# Autodesk Inventor assembly: ensamble_general
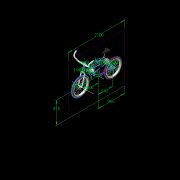
[picture p0: Inventor's stored thumbnail of the model, 180x180]
Saved by Autodesk Inventor 2021 (Build 250183000, 183)
## iProperties
Created: 2021-04-10
Part Number: ensamble_general
Document SubType Name: Assembly
Designer: j2seb
Author: j2seb
## Documents named in this file (10)
- C:\Users\maaro\Documents\UNAL\Automatización de Procesos de Manufactura\Github\Proyecto_APM\02 Inventor\ensamble_general.iam
- C:\Users\maaro\Documents\UNAL\Automatización de Procesos de Manufactura\Github\Proyecto_APM\02 Inventor\Marco_Bicicleta.iam
- C:\Users\maaro\Documents\UNAL\Automatización de Procesos de Manufactura\Github\Proyecto_APM\02 Inventor\Manubrio.ipt
- C:\Users\maaro\Documents\UNAL\Automatización de Procesos de Manufactura\Github\Proyecto_APM\02 Inventor\Ensamble_Llanta.iam
- C:\Users\maaro\Documents\UNAL\Automatización de Procesos de Manufactura\Github\Proyecto_APM\02 Inventor\sillin.iam
- C:\Users\maaro\Documents\UNAL\Automatización de Procesos de Manufactura\Github\Proyecto_APM\02 Inventor\Transmision\Design Accelerator\Roller Chain Sprocket11.ipt
- C:\Users\maaro\Documents\UNAL\Automatización de Procesos de Manufactura\Github\Proyecto_APM\02 Inventor\Transmision\Design Accelerator\Roller Chain Sprocket21.ipt
- C:\Users\maaro\Documents\UNAL\Automatización de Procesos de Manufactura\Github\Proyecto_APM\02 Inventor\Transmision\Design Accelerator\Roller Chain1.ipt
- C:\Users\maaro\Documents\UNAL\Automatización de Procesos de Manufactura\Github\Proyecto_APM\02 Inventor\Transmision\Eslabón 1.ipt
- C:\Users\maaro\Documents\UNAL\Automatización de Procesos de Manufactura\Github\Proyecto_APM\02 Inventor\Transmision\Eslabón 2.ipt
## Components (122 placed, 9 different names)
1. Marco_Bicicleta:1 [sub-assembly] — Coincidencia:2, Coincidencia:3, Flush:1, Cylindrical:2, Mate:5, Mate:6, Mate:8, Mate:10
2. Manubrio:1 — Flush:1, Cylindrical:3, Mate:7, Mate:8
3. Ensamble_Llanta:1 [sub-assembly] — Coincidencia:2
4. Ensamble_Llanta:2 [sub-assembly] — Cylindrical:3
5. sillin:1 [sub-assembly] — Cylindrical:2, Mate:5
6. Roller Chain Sprocket1:1 — Mate:14, Mate:16
7. Roller Chain Sprocket2:1 — Mate:13, Mate:15
8. Roller Chain:1 — Mate:9, Mate:11, Mate:12, Mate:15, Mate:16, Mate:17, Transitional:1, Transitional:2, Transitional:3, Transitional:4, Transitional:5, Transitional:7, Transitional:8, Transitional:9, Transitional:10, Transitional:11, Transitional:12, Transitional:13, Transitional:14, Transitional:15, Transitional:16, Transitional:17, Transitional:18, Transitional:19, Transitional:20, Transitional:21, Transitional:22, Transitional:23, Transitional:24, Transitional:25, Transitional:26, Transitional:27, Transitional:28, Transitional:29, Transitional:30, Transitional:31, Transitional:32, Transitional:33, Transitional:34, Transitional:35, Transitional:36, Transitional:37, Transitional:38, Transitional:39, Transitional:40, Transitional:41, Transitional:42, Transitional:43, Transitional:44, Transitional:45, Transitional:46, Transitional:47, Transitional:48, Transitional:49, Transitional:50, Transitional:51, Transitional:52, Transitional:53, Transitional:54, Transitional:55, Transitional:56, Transitional:57, Transitional:58, Transitional:59, Transitional:60, Transitional:61, Transitional:62, Transitional:63, Transitional:64, Transitional:65, Transitional:66, Transitional:67, Transitional:68, Transitional:69, Transitional:70, Transitional:71, Transitional:72, Transitional:73, Transitional:74, Transitional:75, Transitional:76, Transitional:77, Transitional:78, Transitional:79, Transitional:80, Transitional:81, Transitional:82, Transitional:83, Transitional:84, Transitional:85, Transitional:86, Transitional:87, Transitional:88, Transitional:89, Transitional:90, Transitional:91, Transitional:92, Transitional:93, Transitional:94, Transitional:95, Transitional:96, Transitional:97, Transitional:98, Transitional:99, Transitional:100, Transitional:101, Transitional:102, Transitional:103, Transitional:104, Transitional:105, Transitional:106, Transitional:107, Transitional:108, Transitional:109, Transitional:110, Transitional:111, Transitional:112, Transitional:113, Transitional:114, Transitional:115, Transitional:116, Transitional:117
9. Eslabón 1:1 — Mate:17, Transitional:1, Transitional:2, Mate:18, Mate:19, Mate:20, Mate:21, Mate:22
10. Eslabón 2:1 — Mate:18, Mate:19
11. Eslabón 1:2 — Mate:22, Transitional:3, Transitional:4, Mate:23, Mate:24, Mate:25
12. Eslabón 2:2 — Mate:20, Mate:21, Mate:23
13. Eslabón 1:3 — Mate:26, Transitional:5, Mate:27, Mate:29, Transitional:117
14. Eslabón 2:3 — Mate:24, Mate:25, Mate:26, Mate:27, Mate:28, Mate:30
15. Eslabón 1:4 — Mate:30, Transitional:7, Transitional:8, Mate:31, Mate:33, Transitional:9
16. Eslabón 2:4 — Mate:28, Mate:29, Mate:31, Mate:32
17. Eslabón 1:5 — Mate:34, Transitional:10, Transitional:11, Mate:35, Mate:37
18. Eslabón 2:5 — Mate:32, Mate:33, Mate:34, Mate:35, Mate:36
19. Eslabón 1:6 — Mate:38, Transitional:12, Transitional:13, Mate:39, Mate:41, Transitional:14
20. Eslabón 2:6 — Mate:36, Mate:37, Mate:38, Mate:39, Mate:40
21. Eslabón 1:7 — Mate:42, Transitional:15, Transitional:16, Mate:43, Mate:45
22. Eslabón 2:7 — Mate:40, Mate:41, Mate:42, Mate:43, Mate:44
23. Eslabón 1:8 — Mate:46, Transitional:17, Transitional:18, Mate:47, Mate:49
24. Eslabón 2:8 — Mate:44, Mate:45, Mate:46, Mate:47, Mate:48
25. Eslabón 1:9 — Mate:50, Transitional:19, Transitional:20, Mate:51, Mate:53
26. Eslabón 2:9 — Mate:48, Mate:49, Mate:50, Mate:51, Mate:52
27. Eslabón 1:10 — Mate:54, Transitional:21, Transitional:22, Mate:55, Mate:57
28. Eslabón 2:10 — Mate:52, Mate:53, Mate:54, Mate:55, Mate:56
29. Eslabón 1:11 — Mate:58, Transitional:23, Transitional:24, Mate:59, Mate:61
30. Eslabón 2:11 — Mate:56, Mate:57, Mate:58, Mate:59, Mate:60
31. Eslabón 1:12 — Mate:62, Transitional:25, Transitional:26, Mate:63, Mate:65
32. Eslabón 2:12 — Mate:60, Mate:61, Mate:62, Mate:63, Mate:64
33. Eslabón 1:13 — Mate:66, Transitional:27, Transitional:28, Mate:67, Mate:69
34. Eslabón 2:13 — Mate:64, Mate:65, Mate:66, Mate:67, Mate:68
35. Eslabón 1:14 — Mate:70, Transitional:29, Transitional:30, Mate:71, Mate:73
36. Eslabón 2:14 — Mate:68, Mate:69, Mate:70, Mate:71, Mate:72
37. Eslabón 1:15 — Mate:74, Transitional:31, Transitional:32, Mate:75, Mate:77
38. Eslabón 2:15 — Mate:72, Mate:73, Mate:74, Mate:75, Mate:76
39. Eslabón 1:16 — Mate:78, Transitional:33, Transitional:34, Mate:79, Mate:81
40. Eslabón 2:16 — Mate:76, Mate:77, Mate:78, Mate:79, Mate:80
41. Eslabón 1:17 — Mate:82, Mate:83, Transitional:35, Transitional:36, Mate:85
42. Eslabón 2:17 — Mate:80, Mate:81, Mate:82, Mate:83, Mate:84
43. Eslabón 1:18 — Mate:86, Mate:87, Transitional:37, Transitional:38, Mate:89
44. Eslabón 2:18 — Mate:84, Mate:85, Mate:86, Mate:87, Mate:88
45. Eslabón 1:19 — Mate:90, Mate:91, Transitional:39, Transitional:40, Mate:93
46. Eslabón 2:19 — Mate:88, Mate:89, Mate:90, Mate:91, Mate:92
47. Eslabón 1:20 — Mate:94, Mate:95, Transitional:41, Transitional:42, Mate:97
48. Eslabón 2:20 — Mate:92, Mate:93, Mate:94, Mate:95, Mate:96
49. Eslabón 1:21 — Mate:98, Mate:99, Transitional:43, Transitional:44, Mate:101
50. Eslabón 2:21 — Mate:96, Mate:97, Mate:98, Mate:99, Mate:100
51. Eslabón 1:22 — Mate:102, Mate:103, Transitional:45, Transitional:46, Mate:105
52. Eslabón 2:22 — Mate:100, Mate:101, Mate:102, Mate:103, Mate:104
53. Eslabón 1:23 — Mate:106, Mate:107, Transitional:47, Transitional:48, Mate:109
54. Eslabón 2:23 — Mate:104, Mate:105, Mate:106, Mate:107, Mate:108
55. Eslabón 1:24 — Mate:110, Mate:111, Transitional:49, Transitional:50, Mate:113
56. Eslabón 2:24 — Mate:108, Mate:109, Mate:110, Mate:111, Mate:112
57. Eslabón 1:25 — Mate:114, Mate:115, Transitional:51, Transitional:52, Mate:117
58. Eslabón 2:25 — Mate:112, Mate:113, Mate:114, Mate:115, Mate:116
59. Eslabón 1:26 — Mate:118, Mate:119, Transitional:53, Transitional:54, Mate:121
60. Eslabón 2:26 — Mate:116, Mate:117, Mate:118, Mate:119, Mate:120
61. Eslabón 1:27 — Mate:122, Mate:123, Transitional:55, Transitional:56, Mate:125
62. Eslabón 2:27 — Mate:120, Mate:121, Mate:122, Mate:123, Mate:124
63. Eslabón 1:28 — Mate:126, Mate:127, Transitional:57, Transitional:58, Mate:129
64. Eslabón 2:28 — Mate:124, Mate:125, Mate:126, Mate:127, Mate:128
65. Eslabón 1:29 — Mate:130, Mate:131, Transitional:59, Transitional:60, Mate:133
66. Eslabón 2:29 — Mate:128, Mate:129, Mate:130, Mate:131, Mate:132
67. Eslabón 1:30 — Mate:134, Transitional:61, Transitional:62, Mate:135, Mate:137
68. Eslabón 2:30 — Mate:132, Mate:133, Mate:134, Mate:135, Mate:136
69. Eslabón 1:31 — Mate:138, Mate:139, Transitional:63, Transitional:64, Mate:141
70. Eslabón 2:31 — Mate:136, Mate:137, Mate:138, Mate:139, Mate:140
71. Eslabón 1:32 — Mate:142, Transitional:65, Transitional:66, Mate:143, Mate:145
72. Eslabón 2:32 — Mate:140, Mate:141, Mate:142, Mate:143, Mate:144
73. Eslabón 1:33 — Mate:146, Transitional:67, Transitional:68, Mate:147, Mate:149
74. Eslabón 2:33 — Mate:144, Mate:145, Mate:146, Mate:147, Mate:148
75. Eslabón 1:34 — Mate:150, Transitional:69, Transitional:70, Mate:151, Mate:153
76. Eslabón 2:34 — Mate:148, Mate:149, Mate:150, Mate:151, Mate:152
77. Eslabón 1:35 — Mate:154, Mate:155, Transitional:71, Transitional:72, Mate:157
78. Eslabón 2:35 — Mate:152, Mate:153, Mate:154, Mate:155, Mate:156
79. Eslabón 1:36 — Mate:158, Mate:159, Transitional:73, Transitional:74, Mate:161
80. Eslabón 2:36 — Mate:156, Mate:157, Mate:158, Mate:159, Mate:160
81. Eslabón 1:37 — Mate:162, Mate:163, Transitional:75, Transitional:76, Mate:165
82. Eslabón 2:37 — Mate:160, Mate:161, Mate:162, Mate:163, Mate:164
83. Eslabón 1:38 — Mate:166, Mate:167, Transitional:77, Transitional:78, Mate:169
84. Eslabón 2:38 — Mate:164, Mate:165, Mate:166, Mate:167, Mate:168
85. Eslabón 1:39 — Mate:170, Mate:171, Transitional:79, Transitional:80, Mate:173
86. Eslabón 2:39 — Mate:168, Mate:169, Mate:170, Mate:171, Mate:172
87. Eslabón 1:40 — Mate:174, Mate:175, Transitional:81, Transitional:82, Mate:177
88. Eslabón 2:40 — Mate:172, Mate:173, Mate:174, Mate:175, Mate:176
89. Eslabón 1:41 — Mate:178, Mate:179, Transitional:83, Transitional:84, Mate:181
90. Eslabón 2:41 — Mate:176, Mate:177, Mate:178, Mate:179, Mate:180
91. Eslabón 1:42 — Mate:182, Mate:183, Transitional:85, Transitional:86, Mate:185
92. Eslabón 2:42 — Mate:180, Mate:181, Mate:182, Mate:183, Mate:184
93. Eslabón 1:43 — Mate:186, Mate:187, Transitional:87, Transitional:88, Mate:189
94. Eslabón 2:43 — Mate:184, Mate:185, Mate:186, Mate:187, Mate:188
95. Eslabón 1:44 — Mate:190, Mate:191, Transitional:89, Transitional:90, Mate:193
96. Eslabón 2:44 — Mate:188, Mate:189, Mate:190, Mate:191, Mate:192
97. Eslabón 1:45 — Mate:194, Mate:195, Transitional:91, Transitional:92, Mate:197
98. Eslabón 2:45 — Mate:192, Mate:193, Mate:194, Mate:195, Mate:196
99. Eslabón 1:46 — Mate:198, Mate:199, Transitional:93, Transitional:94, Mate:201
100. Eslabón 2:46 — Mate:196, Mate:197, Mate:198, Mate:199, Mate:200
101. Eslabón 1:47 — Mate:202, Mate:203, Transitional:95, Transitional:96, Mate:205
102. Eslabón 2:47 — Mate:200, Mate:201, Mate:202, Mate:203, Mate:204
103. Eslabón 1:48 — Mate:206, Mate:207, Transitional:97, Transitional:98, Mate:209
104. Eslabón 2:48 — Mate:204, Mate:205, Mate:206, Mate:207, Mate:208
105. Eslabón 1:49 — Mate:210, Mate:211, Transitional:99, Transitional:100, Mate:213
106. Eslabón 2:49 — Mate:208, Mate:209, Mate:210, Mate:211, Mate:212
107. Eslabón 1:50 — Mate:214, Mate:215, Transitional:101, Transitional:102, Mate:217
108. Eslabón 2:50 — Mate:212, Mate:213, Mate:214, Mate:215, Mate:216
109. Eslabón 1:51 — Mate:218, Mate:219, Transitional:103, Transitional:104, Mate:221
110. Eslabón 2:51 — Mate:216, Mate:217, Mate:218, Mate:219, Mate:220
111. Eslabón 1:52 — Mate:222, Mate:223, Transitional:105, Transitional:106, Mate:225
112. Eslabón 2:52 — Mate:220, Mate:221, Mate:222, Mate:223, Mate:224
113. Eslabón 1:53 — Mate:226, Mate:227, Transitional:107, Transitional:108, Mate:229
114. Eslabón 2:53 — Mate:224, Mate:225, Mate:226, Mate:227, Mate:228
115. Eslabón 1:54 — Mate:230, Mate:231, Transitional:109, Transitional:110, Mate:233
116. Eslabón 2:54 — Mate:228, Mate:229, Mate:230, Mate:231, Mate:232
117. Eslabón 1:55 — Mate:234, Mate:235, Transitional:111, Transitional:112, Mate:237
118. Eslabón 2:55 — Mate:232, Mate:233, Mate:234, Mate:235, Mate:236
119. Eslabón 1:56 — Mate:238, Mate:239, Transitional:113, Transitional:114, Mate:241
120. Eslabón 2:56 — Mate:236, Mate:237, Mate:238, Mate:239, Mate:240
121. Eslabón 1:57 — Mate:242, Mate:243, Transitional:115, Transitional:116
122. Eslabón 2:57 — Mate:240, Mate:241, Mate:242, Mate:243
## Relationships (361: Mate 241, Transitional 116, CylindricalJoint 2, Angle 1, Flush 1)
- Coincidencia:2 [Mate]: Marco_Bicicleta:1 ↔ Ensamble_Llanta:1
- Coincidencia:3 [Mate]: Marco_Bicicleta:1
- Ángulo:1 [Angle] (0 deg)
- Flush:1 (-55.052 mm): Marco_Bicicleta:1 ↔ Manubrio:1
- Cylindrical:2: Marco_Bicicleta:1 ↔ sillin:1
- Mate:5 (-50 mm): Marco_Bicicleta:1 ↔ sillin:1
- Cylindrical:3: Manubrio:1 ↔ Ensamble_Llanta:2
- Mate:6: Marco_Bicicleta:1
- Mate:7: Manubrio:1
- Mate:8: Marco_Bicicleta:1 ↔ Manubrio:1
- Mate:9: Roller Chain:1
- Mate:10: Marco_Bicicleta:1
- Mate:11: Roller Chain:1
- Mate:12: Roller Chain:1
- Mate:13: Roller Chain Sprocket2:1
- Mate:14: Roller Chain Sprocket1:1
- Mate:15: Roller Chain Sprocket2:1 ↔ Roller Chain:1
- Mate:16: Roller Chain Sprocket1:1 ↔ Roller Chain:1
- Mate:17: Roller Chain:1 ↔ Eslabón 1:1
- Transitional:1: Roller Chain:1 ↔ Eslabón 1:1
- Transitional:2: Roller Chain:1 ↔ Eslabón 1:1
- Mate:18: Eslabón 1:1 ↔ Eslabón 2:1
- Mate:19: Eslabón 1:1 ↔ Eslabón 2:1
- Mate:20: Eslabón 1:1 ↔ Eslabón 2:2
- Mate:21: Eslabón 1:1 ↔ Eslabón 2:2
- Mate:22: Eslabón 1:1 ↔ Eslabón 1:2
- Transitional:3: Roller Chain:1 ↔ Eslabón 1:2
- Transitional:4: Roller Chain:1 ↔ Eslabón 1:2
- Mate:23: Eslabón 1:2 ↔ Eslabón 2:2
- Mate:24: Eslabón 1:2 ↔ Eslabón 2:3
- Mate:25: Eslabón 1:2 ↔ Eslabón 2:3
- Mate:26: Eslabón 1:3 ↔ Eslabón 2:3
- Transitional:5: Roller Chain:1 ↔ Eslabón 1:3
- Mate:27: Eslabón 1:3 ↔ Eslabón 2:3
- Mate:28: Eslabón 2:3 ↔ Eslabón 2:4
- Mate:29: Eslabón 1:3 ↔ Eslabón 2:4
- Mate:30: Eslabón 2:3 ↔ Eslabón 1:4
- Transitional:7: Roller Chain:1 ↔ Eslabón 1:4
- Transitional:8: Roller Chain:1 ↔ Eslabón 1:4
- Mate:31: Eslabón 1:4 ↔ Eslabón 2:4
- Mate:32: Eslabón 2:4 ↔ Eslabón 2:5
- Mate:33: Eslabón 1:4 ↔ Eslabón 2:5
- Mate:34: Eslabón 1:5 ↔ Eslabón 2:5
- Transitional:9: Roller Chain:1 ↔ Eslabón 1:4
- Transitional:10: Roller Chain:1 ↔ Eslabón 1:5
- Transitional:11: Roller Chain:1 ↔ Eslabón 1:5
- Mate:35: Eslabón 1:5 ↔ Eslabón 2:5
- Mate:36: Eslabón 2:5 ↔ Eslabón 2:6
- Mate:37: Eslabón 1:5 ↔ Eslabón 2:6
- Mate:38: Eslabón 1:6 ↔ Eslabón 2:6
- Transitional:12: Roller Chain:1 ↔ Eslabón 1:6
- Transitional:13: Roller Chain:1 ↔ Eslabón 1:6
- Mate:39: Eslabón 1:6 ↔ Eslabón 2:6
- Mate:40: Eslabón 2:6 ↔ Eslabón 2:7
- Mate:41: Eslabón 1:6 ↔ Eslabón 2:7
- Mate:42: Eslabón 1:7 ↔ Eslabón 2:7
- Transitional:14: Roller Chain:1 ↔ Eslabón 1:6
- Transitional:15: Roller Chain:1 ↔ Eslabón 1:7
- Transitional:16: Roller Chain:1 ↔ Eslabón 1:7
- Mate:43: Eslabón 1:7 ↔ Eslabón 2:7
- Mate:44: Eslabón 2:7 ↔ Eslabón 2:8
- Mate:45: Eslabón 1:7 ↔ Eslabón 2:8
- Mate:46: Eslabón 1:8 ↔ Eslabón 2:8
- Transitional:17: Roller Chain:1 ↔ Eslabón 1:8
- Transitional:18: Roller Chain:1 ↔ Eslabón 1:8
- Mate:47: Eslabón 1:8 ↔ Eslabón 2:8
- Mate:48: Eslabón 2:8 ↔ Eslabón 2:9
- Mate:49: Eslabón 1:8 ↔ Eslabón 2:9
- Mate:50: Eslabón 1:9 ↔ Eslabón 2:9
- Transitional:19: Roller Chain:1 ↔ Eslabón 1:9
- Transitional:20: Roller Chain:1 ↔ Eslabón 1:9
- Mate:51: Eslabón 1:9 ↔ Eslabón 2:9
- Mate:52: Eslabón 2:9 ↔ Eslabón 2:10
- Mate:53: Eslabón 1:9 ↔ Eslabón 2:10
- Mate:54: Eslabón 1:10 ↔ Eslabón 2:10
- Transitional:21: Roller Chain:1 ↔ Eslabón 1:10
- Transitional:22: Roller Chain:1 ↔ Eslabón 1:10
- Mate:55: Eslabón 1:10 ↔ Eslabón 2:10
- Mate:56: Eslabón 2:10 ↔ Eslabón 2:11
- Mate:57: Eslabón 1:10 ↔ Eslabón 2:11
- Mate:58: Eslabón 1:11 ↔ Eslabón 2:11
- Transitional:23: Roller Chain:1 ↔ Eslabón 1:11
- Transitional:24: Roller Chain:1 ↔ Eslabón 1:11
- Mate:59: Eslabón 1:11 ↔ Eslabón 2:11
- Mate:60: Eslabón 2:11 ↔ Eslabón 2:12
- Mate:61: Eslabón 1:11 ↔ Eslabón 2:12
- Mate:62: Eslabón 1:12 ↔ Eslabón 2:12
- Transitional:25: Roller Chain:1 ↔ Eslabón 1:12
- Transitional:26: Roller Chain:1 ↔ Eslabón 1:12
- Mate:63: Eslabón 1:12 ↔ Eslabón 2:12
- Mate:64: Eslabón 2:12 ↔ Eslabón 2:13
- Mate:65: Eslabón 1:12 ↔ Eslabón 2:13
- Mate:66: Eslabón 1:13 ↔ Eslabón 2:13
- Transitional:27: Roller Chain:1 ↔ Eslabón 1:13
- Transitional:28: Roller Chain:1 ↔ Eslabón 1:13
- Mate:67: Eslabón 1:13 ↔ Eslabón 2:13
- Mate:68: Eslabón 2:13 ↔ Eslabón 2:14
- Mate:69: Eslabón 1:13 ↔ Eslabón 2:14
- Mate:70: Eslabón 1:14 ↔ Eslabón 2:14
- Transitional:29: Roller Chain:1 ↔ Eslabón 1:14
- Transitional:30: Roller Chain:1 ↔ Eslabón 1:14
- Mate:71: Eslabón 1:14 ↔ Eslabón 2:14
- Mate:72: Eslabón 2:14 ↔ Eslabón 2:15
- Mate:73: Eslabón 1:14 ↔ Eslabón 2:15
- Mate:74: Eslabón 1:15 ↔ Eslabón 2:15
- Transitional:31: Roller Chain:1 ↔ Eslabón 1:15
- Transitional:32: Roller Chain:1 ↔ Eslabón 1:15
- Mate:75: Eslabón 1:15 ↔ Eslabón 2:15
- Mate:76: Eslabón 2:15 ↔ Eslabón 2:16
- Mate:77: Eslabón 1:15 ↔ Eslabón 2:16
- Mate:78: Eslabón 1:16 ↔ Eslabón 2:16
- Transitional:33: Roller Chain:1 ↔ Eslabón 1:16
- Transitional:34: Roller Chain:1 ↔ Eslabón 1:16
- Mate:79: Eslabón 1:16 ↔ Eslabón 2:16
- Mate:80: Eslabón 2:16 ↔ Eslabón 2:17
- Mate:81: Eslabón 1:16 ↔ Eslabón 2:17
- Mate:82: Eslabón 1:17 ↔ Eslabón 2:17
- Mate:83: Eslabón 1:17 ↔ Eslabón 2:17
- Transitional:35: Roller Chain:1 ↔ Eslabón 1:17
- Transitional:36: Roller Chain:1 ↔ Eslabón 1:17
- Mate:84: Eslabón 2:17 ↔ Eslabón 2:18
- Mate:85: Eslabón 1:17 ↔ Eslabón 2:18
- Mate:86: Eslabón 1:18 ↔ Eslabón 2:18
- Mate:87: Eslabón 1:18 ↔ Eslabón 2:18
- Transitional:37: Roller Chain:1 ↔ Eslabón 1:18
- Transitional:38: Roller Chain:1 ↔ Eslabón 1:18
- Mate:88: Eslabón 2:18 ↔ Eslabón 2:19
- Mate:89: Eslabón 1:18 ↔ Eslabón 2:19
- Mate:90: Eslabón 1:19 ↔ Eslabón 2:19
- Mate:91: Eslabón 1:19 ↔ Eslabón 2:19
- Transitional:39: Roller Chain:1 ↔ Eslabón 1:19
- Transitional:40: Roller Chain:1 ↔ Eslabón 1:19
- Mate:92: Eslabón 2:19 ↔ Eslabón 2:20
- Mate:93: Eslabón 1:19 ↔ Eslabón 2:20
- Mate:94: Eslabón 1:20 ↔ Eslabón 2:20
- Mate:95: Eslabón 1:20 ↔ Eslabón 2:20
- Transitional:41: Roller Chain:1 ↔ Eslabón 1:20
- Transitional:42: Roller Chain:1 ↔ Eslabón 1:20
- Mate:96: Eslabón 2:20 ↔ Eslabón 2:21
- Mate:97: Eslabón 1:20 ↔ Eslabón 2:21
- Mate:98: Eslabón 1:21 ↔ Eslabón 2:21
- Mate:99: Eslabón 1:21 ↔ Eslabón 2:21
- Transitional:43: Roller Chain:1 ↔ Eslabón 1:21
- Transitional:44: Roller Chain:1 ↔ Eslabón 1:21
- Mate:100: Eslabón 2:21 ↔ Eslabón 2:22
- Mate:101: Eslabón 1:21 ↔ Eslabón 2:22
- Mate:102: Eslabón 1:22 ↔ Eslabón 2:22
- Mate:103: Eslabón 1:22 ↔ Eslabón 2:22
- Transitional:45: Roller Chain:1 ↔ Eslabón 1:22
- Transitional:46: Roller Chain:1 ↔ Eslabón 1:22
- Mate:104: Eslabón 2:22 ↔ Eslabón 2:23
- Mate:105: Eslabón 1:22 ↔ Eslabón 2:23
- Mate:106: Eslabón 1:23 ↔ Eslabón 2:23
- Mate:107: Eslabón 1:23 ↔ Eslabón 2:23
- Transitional:47: Roller Chain:1 ↔ Eslabón 1:23
- Transitional:48: Roller Chain:1 ↔ Eslabón 1:23
- Mate:108: Eslabón 2:23 ↔ Eslabón 2:24
- Mate:109: Eslabón 1:23 ↔ Eslabón 2:24
- Mate:110: Eslabón 1:24 ↔ Eslabón 2:24
- Mate:111: Eslabón 1:24 ↔ Eslabón 2:24
- Transitional:49: Roller Chain:1 ↔ Eslabón 1:24
- Transitional:50: Roller Chain:1 ↔ Eslabón 1:24
- Mate:112: Eslabón 2:24 ↔ Eslabón 2:25
- Mate:113: Eslabón 1:24 ↔ Eslabón 2:25
- Mate:114: Eslabón 1:25 ↔ Eslabón 2:25
- Mate:115: Eslabón 1:25 ↔ Eslabón 2:25
- Transitional:51: Roller Chain:1 ↔ Eslabón 1:25
- Transitional:52: Roller Chain:1 ↔ Eslabón 1:25
- Mate:116: Eslabón 2:25 ↔ Eslabón 2:26
- Mate:117: Eslabón 1:25 ↔ Eslabón 2:26
- Mate:118: Eslabón 1:26 ↔ Eslabón 2:26
- Mate:119: Eslabón 1:26 ↔ Eslabón 2:26
- Transitional:53: Roller Chain:1 ↔ Eslabón 1:26
- Transitional:54: Roller Chain:1 ↔ Eslabón 1:26
- Mate:120: Eslabón 2:26 ↔ Eslabón 2:27
- Mate:121: Eslabón 1:26 ↔ Eslabón 2:27
- Mate:122: Eslabón 1:27 ↔ Eslabón 2:27
- Mate:123: Eslabón 1:27 ↔ Eslabón 2:27
- Transitional:55: Roller Chain:1 ↔ Eslabón 1:27
- Transitional:56: Roller Chain:1 ↔ Eslabón 1:27
- Mate:124: Eslabón 2:27 ↔ Eslabón 2:28
- Mate:125: Eslabón 1:27 ↔ Eslabón 2:28
- Mate:126: Eslabón 1:28 ↔ Eslabón 2:28
- Mate:127: Eslabón 1:28 ↔ Eslabón 2:28
- Transitional:57: Roller Chain:1 ↔ Eslabón 1:28
- Transitional:58: Roller Chain:1 ↔ Eslabón 1:28
- Mate:128: Eslabón 2:28 ↔ Eslabón 2:29
- Mate:129: Eslabón 1:28 ↔ Eslabón 2:29
- Mate:130: Eslabón 1:29 ↔ Eslabón 2:29
- Mate:131: Eslabón 1:29 ↔ Eslabón 2:29
- Transitional:59: Roller Chain:1 ↔ Eslabón 1:29
- Transitional:60: Roller Chain:1 ↔ Eslabón 1:29
- Mate:132: Eslabón 2:29 ↔ Eslabón 2:30
- Mate:133: Eslabón 1:29 ↔ Eslabón 2:30
- Mate:134: Eslabón 1:30 ↔ Eslabón 2:30
- Transitional:61: Roller Chain:1 ↔ Eslabón 1:30
- Transitional:62: Roller Chain:1 ↔ Eslabón 1:30
- Mate:135: Eslabón 1:30 ↔ Eslabón 2:30
- Mate:136: Eslabón 2:30 ↔ Eslabón 2:31
- Mate:137: Eslabón 1:30 ↔ Eslabón 2:31
- Mate:138: Eslabón 1:31 ↔ Eslabón 2:31
- Mate:139: Eslabón 1:31 ↔ Eslabón 2:31
- Transitional:63: Roller Chain:1 ↔ Eslabón 1:31
- Transitional:64: Roller Chain:1 ↔ Eslabón 1:31
- Mate:140: Eslabón 2:31 ↔ Eslabón 2:32
- Mate:141: Eslabón 1:31 ↔ Eslabón 2:32
- Mate:142: Eslabón 1:32 ↔ Eslabón 2:32
- Transitional:65: Roller Chain:1 ↔ Eslabón 1:32
- Transitional:66: Roller Chain:1 ↔ Eslabón 1:32
- Mate:143: Eslabón 1:32 ↔ Eslabón 2:32
- Mate:144: Eslabón 2:32 ↔ Eslabón 2:33
- Mate:145: Eslabón 1:32 ↔ Eslabón 2:33
- Mate:146: Eslabón 1:33 ↔ Eslabón 2:33
- Transitional:67: Roller Chain:1 ↔ Eslabón 1:33
- Transitional:68: Roller Chain:1 ↔ Eslabón 1:33
- Mate:147: Eslabón 1:33 ↔ Eslabón 2:33
- Mate:148: Eslabón 2:33 ↔ Eslabón 2:34
- Mate:149: Eslabón 1:33 ↔ Eslabón 2:34
- Mate:150: Eslabón 1:34 ↔ Eslabón 2:34
- Transitional:69: Roller Chain:1 ↔ Eslabón 1:34
- Transitional:70: Roller Chain:1 ↔ Eslabón 1:34
- Mate:151: Eslabón 1:34 ↔ Eslabón 2:34
- Mate:152: Eslabón 2:34 ↔ Eslabón 2:35
- Mate:153: Eslabón 1:34 ↔ Eslabón 2:35
- Mate:154: Eslabón 1:35 ↔ Eslabón 2:35
- Mate:155: Eslabón 1:35 ↔ Eslabón 2:35
- Transitional:71: Roller Chain:1 ↔ Eslabón 1:35
- Transitional:72: Roller Chain:1 ↔ Eslabón 1:35
- Mate:156: Eslabón 2:35 ↔ Eslabón 2:36
- Mate:157: Eslabón 1:35 ↔ Eslabón 2:36
- Mate:158: Eslabón 1:36 ↔ Eslabón 2:36
- Mate:159: Eslabón 1:36 ↔ Eslabón 2:36
- Transitional:73: Roller Chain:1 ↔ Eslabón 1:36
- Transitional:74: Roller Chain:1 ↔ Eslabón 1:36
- Mate:160: Eslabón 2:36 ↔ Eslabón 2:37
- Mate:161: Eslabón 1:36 ↔ Eslabón 2:37
- Mate:162: Eslabón 1:37 ↔ Eslabón 2:37
- Mate:163: Eslabón 1:37 ↔ Eslabón 2:37
- Transitional:75: Roller Chain:1 ↔ Eslabón 1:37
- Transitional:76: Roller Chain:1 ↔ Eslabón 1:37
- Mate:164: Eslabón 2:37 ↔ Eslabón 2:38
- Mate:165: Eslabón 1:37 ↔ Eslabón 2:38
- Mate:166: Eslabón 1:38 ↔ Eslabón 2:38
- Mate:167: Eslabón 1:38 ↔ Eslabón 2:38
- Transitional:77: Roller Chain:1 ↔ Eslabón 1:38
- Transitional:78: Roller Chain:1 ↔ Eslabón 1:38
- Mate:168: Eslabón 2:38 ↔ Eslabón 2:39
- Mate:169: Eslabón 1:38 ↔ Eslabón 2:39
- Mate:170: Eslabón 1:39 ↔ Eslabón 2:39
- Mate:171: Eslabón 1:39 ↔ Eslabón 2:39
- Transitional:79: Roller Chain:1 ↔ Eslabón 1:39
- Transitional:80: Roller Chain:1 ↔ Eslabón 1:39
- Mate:172: Eslabón 2:39 ↔ Eslabón 2:40
- Mate:173: Eslabón 1:39 ↔ Eslabón 2:40
- Mate:174: Eslabón 1:40 ↔ Eslabón 2:40
- Mate:175: Eslabón 1:40 ↔ Eslabón 2:40
- Transitional:81: Roller Chain:1 ↔ Eslabón 1:40
- Transitional:82: Roller Chain:1 ↔ Eslabón 1:40
- Mate:176: Eslabón 2:40 ↔ Eslabón 2:41
- Mate:177: Eslabón 1:40 ↔ Eslabón 2:41
- Mate:178: Eslabón 1:41 ↔ Eslabón 2:41
- Mate:179: Eslabón 1:41 ↔ Eslabón 2:41
- Transitional:83: Roller Chain:1 ↔ Eslabón 1:41
- Transitional:84: Roller Chain:1 ↔ Eslabón 1:41
- Mate:180: Eslabón 2:41 ↔ Eslabón 2:42
- Mate:181: Eslabón 1:41 ↔ Eslabón 2:42
- Mate:182: Eslabón 1:42 ↔ Eslabón 2:42
- Mate:183: Eslabón 1:42 ↔ Eslabón 2:42
- Transitional:85: Roller Chain:1 ↔ Eslabón 1:42
- Transitional:86: Roller Chain:1 ↔ Eslabón 1:42
- Mate:184: Eslabón 2:42 ↔ Eslabón 2:43
- Mate:185: Eslabón 1:42 ↔ Eslabón 2:43
- Mate:186: Eslabón 1:43 ↔ Eslabón 2:43
- Mate:187: Eslabón 1:43 ↔ Eslabón 2:43
- Transitional:87: Roller Chain:1 ↔ Eslabón 1:43
- Transitional:88: Roller Chain:1 ↔ Eslabón 1:43
- Mate:188: Eslabón 2:43 ↔ Eslabón 2:44
- Mate:189: Eslabón 1:43 ↔ Eslabón 2:44
- Mate:190: Eslabón 1:44 ↔ Eslabón 2:44
- Mate:191: Eslabón 1:44 ↔ Eslabón 2:44
- Transitional:89: Roller Chain:1 ↔ Eslabón 1:44
- Transitional:90: Roller Chain:1 ↔ Eslabón 1:44
- Mate:192: Eslabón 2:44 ↔ Eslabón 2:45
- Mate:193: Eslabón 1:44 ↔ Eslabón 2:45
- Mate:194: Eslabón 1:45 ↔ Eslabón 2:45
- Mate:195: Eslabón 1:45 ↔ Eslabón 2:45
- Transitional:91: Roller Chain:1 ↔ Eslabón 1:45
- Transitional:92: Roller Chain:1 ↔ Eslabón 1:45
- Mate:196: Eslabón 2:45 ↔ Eslabón 2:46
- Mate:197: Eslabón 1:45 ↔ Eslabón 2:46
- Mate:198: Eslabón 1:46 ↔ Eslabón 2:46
- Mate:199: Eslabón 1:46 ↔ Eslabón 2:46
- Transitional:93: Roller Chain:1 ↔ Eslabón 1:46
- Transitional:94: Roller Chain:1 ↔ Eslabón 1:46
- Mate:200: Eslabón 2:46 ↔ Eslabón 2:47
- Mate:201: Eslabón 1:46 ↔ Eslabón 2:47
- Mate:202: Eslabón 1:47 ↔ Eslabón 2:47
- Mate:203: Eslabón 1:47 ↔ Eslabón 2:47
- Transitional:95: Roller Chain:1 ↔ Eslabón 1:47
- Transitional:96: Roller Chain:1 ↔ Eslabón 1:47
- Mate:204: Eslabón 2:47 ↔ Eslabón 2:48
- Mate:205: Eslabón 1:47 ↔ Eslabón 2:48
- Mate:206: Eslabón 1:48 ↔ Eslabón 2:48
- Mate:207: Eslabón 1:48 ↔ Eslabón 2:48
- Transitional:97: Roller Chain:1 ↔ Eslabón 1:48
- Transitional:98: Roller Chain:1 ↔ Eslabón 1:48
- Mate:208: Eslabón 2:48 ↔ Eslabón 2:49
- Mate:209: Eslabón 1:48 ↔ Eslabón 2:49
- Mate:210: Eslabón 1:49 ↔ Eslabón 2:49
- Mate:211: Eslabón 1:49 ↔ Eslabón 2:49
- Transitional:99: Roller Chain:1 ↔ Eslabón 1:49
- Transitional:100: Roller Chain:1 ↔ Eslabón 1:49
- Mate:212: Eslabón 2:49 ↔ Eslabón 2:50
- Mate:213: Eslabón 1:49 ↔ Eslabón 2:50
- Mate:214: Eslabón 1:50 ↔ Eslabón 2:50
- Mate:215: Eslabón 1:50 ↔ Eslabón 2:50
- Transitional:101: Roller Chain:1 ↔ Eslabón 1:50
- Transitional:102: Roller Chain:1 ↔ Eslabón 1:50
- Mate:216: Eslabón 2:50 ↔ Eslabón 2:51
- Mate:217: Eslabón 1:50 ↔ Eslabón 2:51
- Mate:218: Eslabón 1:51 ↔ Eslabón 2:51
- Mate:219: Eslabón 1:51 ↔ Eslabón 2:51
- Transitional:103: Roller Chain:1 ↔ Eslabón 1:51
- Transitional:104: Roller Chain:1 ↔ Eslabón 1:51
- Mate:220: Eslabón 2:51 ↔ Eslabón 2:52
- Mate:221: Eslabón 1:51 ↔ Eslabón 2:52
- Mate:222: Eslabón 1:52 ↔ Eslabón 2:52
- Mate:223: Eslabón 1:52 ↔ Eslabón 2:52
- Transitional:105: Roller Chain:1 ↔ Eslabón 1:52
- Transitional:106: Roller Chain:1 ↔ Eslabón 1:52
- Mate:224: Eslabón 2:52 ↔ Eslabón 2:53
- Mate:225: Eslabón 1:52 ↔ Eslabón 2:53
- Mate:226: Eslabón 1:53 ↔ Eslabón 2:53
- Mate:227: Eslabón 1:53 ↔ Eslabón 2:53
- Transitional:107: Roller Chain:1 ↔ Eslabón 1:53
- Transitional:108: Roller Chain:1 ↔ Eslabón 1:53
- Mate:228: Eslabón 2:53 ↔ Eslabón 2:54
- Mate:229: Eslabón 1:53 ↔ Eslabón 2:54
- Mate:230: Eslabón 1:54 ↔ Eslabón 2:54
- Mate:231: Eslabón 1:54 ↔ Eslabón 2:54
- Transitional:109: Roller Chain:1 ↔ Eslabón 1:54
- Transitional:110: Roller Chain:1 ↔ Eslabón 1:54
- Mate:232: Eslabón 2:54 ↔ Eslabón 2:55
- Mate:233: Eslabón 1:54 ↔ Eslabón 2:55
- Mate:234: Eslabón 1:55 ↔ Eslabón 2:55
- Mate:235: Eslabón 1:55 ↔ Eslabón 2:55
- Transitional:111: Roller Chain:1 ↔ Eslabón 1:55
- Transitional:112: Roller Chain:1 ↔ Eslabón 1:55
- Mate:236: Eslabón 2:55 ↔ Eslabón 2:56
- Mate:237: Eslabón 1:55 ↔ Eslabón 2:56
- Mate:238: Eslabón 1:56 ↔ Eslabón 2:56
- Mate:239: Eslabón 1:56 ↔ Eslabón 2:56
- Transitional:113: Roller Chain:1 ↔ Eslabón 1:56
- Transitional:114: Roller Chain:1 ↔ Eslabón 1:56
- Mate:240: Eslabón 2:56 ↔ Eslabón 2:57
- Mate:241: Eslabón 1:56 ↔ Eslabón 2:57
- Mate:242: Eslabón 1:57 ↔ Eslabón 2:57
- Mate:243: Eslabón 1:57 ↔ Eslabón 2:57
- Transitional:115: Roller Chain:1 ↔ Eslabón 1:57
- Transitional:116: Roller Chain:1 ↔ Eslabón 1:57
- Transitional:117: Roller Chain:1 ↔ Eslabón 1:3
## Named parameters: DExtTub = 42.164 mm, DintTub = 35.052 mm, DIntTubTen = 28 mm, DAguUniMarcoLlanta = 4 mm
